# Autodesk Inventor assembly: link1
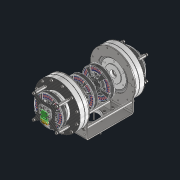
[picture p0: Inventor's stored thumbnail of the model, 180x180]
Saved by Autodesk Inventor 2021 (Build 250183000, 183)
## iProperties
Created: 2021-08-10
Part Number: link1
Document SubType Name: Assembly
Designer: yuta0
Author: yuta0
## Documents named in this file (2)
- C:\Users\yuta0\Documents\GitHub\catchrobo_hardware\mesh\link1.iam
- C:\Users\yuta0\Documents\GitHub\catchrobo_hardware\assy-robot\s-assy-link1.iam
## Components (1 placed, 1 different names)
1. s-assy-link1:1 [sub-assembly] — メイト:2, メイト:3
## Relationships (2: Mate 2)
- メイト:2 [Mate]: s-assy-link1:1
- メイト:3 [Mate]: s-assy-link1:1
